# Autodesk Inventor assembly: inner_glide_cartrige_full_assembly
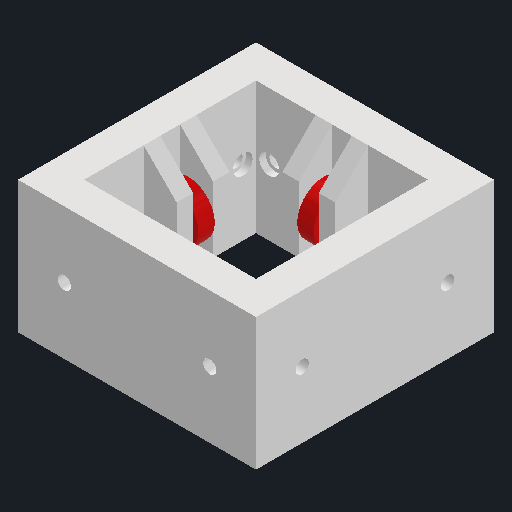
[picture p0: Inventor's stored thumbnail of the model, 512x512]
Saved by Autodesk Inventor 2024 (Build 280153000, 153)
## iProperties
Created: 2023-05-23
Part Number: inner_glide_cartrige_full_assembly
Document SubType Name: Assembly
Designer: aasmu
Author: aasmu
## Documents named in this file (4)
- C:\Users\aasmu\Documents\standing_desk\inner_glide_cartrige_full_assembly.iam
- C:\Users\aasmu\Documents\standing_desk\inner_glide_cartrige.ipt
- C:\Users\aasmu\Documents\standing_desk\4_ball_bearing.ipt
- C:\Users\aasmu\Documents\standing_desk\ball_bearing_rod.ipt
## Components (9 placed, 3 different names)
1. inner_glide_cartrige:1 — Rotational:1, Rotational:2, Rotational:3, Rotational:4
2. 4_ball_bearing:1 — Cylindrical:1
3. 4_ball_bearing:2 — Cylindrical:3
4. 4_ball_bearing:3 — Cylindrical:4
5. 4_ball_bearing:4 — Cylindrical:2
6. ball_bearing_rod:1 — Cylindrical:4, Rotational:4
7. ball_bearing_rod:2 — Cylindrical:2, Rotational:3
8. ball_bearing_rod:3 — Cylindrical:3, Rotational:1
9. ball_bearing_rod:4 — Cylindrical:1, Rotational:2
## Relationships (8: CylindricalJoint 4, RevoluteJoint 4)
- Cylindrical:1: 4_ball_bearing:1 ↔ ball_bearing_rod:4
- Cylindrical:2: 4_ball_bearing:4 ↔ ball_bearing_rod:2
- Cylindrical:3: 4_ball_bearing:2 ↔ ball_bearing_rod:3
- Cylindrical:4: 4_ball_bearing:3 ↔ ball_bearing_rod:1
- Rotational:1 [RevoluteJoint]: inner_glide_cartrige:1 ↔ ball_bearing_rod:3
- Rotational:2 [RevoluteJoint]: inner_glide_cartrige:1 ↔ ball_bearing_rod:4
- Rotational:3 [RevoluteJoint]: inner_glide_cartrige:1 ↔ ball_bearing_rod:2
- Rotational:4 [RevoluteJoint]: inner_glide_cartrige:1 ↔ ball_bearing_rod:1
